# Autodesk Inventor assembly: Assembly11 (Cam Sub Assembly)
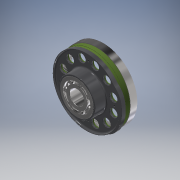
[picture p0: Inventor's stored thumbnail of the model, 180x180]
Saved by Autodesk Inventor 2018 (Build 220112000, 112)
## iProperties
Created: 2023-05-02
Part Number: Assembly11 (Cam Sub Assembly)
Document SubType Name: Assembly
Designer: Habib Mohamed
Author: Habib Mohamed
## Documents named in this file (6)
- D:\Inventor\My projects\Rotary Engine\Assembly\Assembly11 (Cam Sub Assembly).iam
- D:\Inventor\My projects\Rotary Engine\Component 18 (Front Cam Disc).ipt
- D:\Inventor\My projects\Rotary Engine\Component 19 (Rear Cam Disc).ipt
- D:\Inventor\My projects\Rotary Engine\Component 21 (Hollow Wheel).ipt
- C:\Users\Habib Mohamed\Documents\Inventor\Content Center Files\R2018\en-US\DIN 625 - T3\DIN 625 T3 - 4202 - 15 x 35 x 14.ipt
- C:\Users\Habib Mohamed\Documents\Inventor\Content Center Files\R2018\en-US\ISO 7046-1(2)\DIN EN ISO 7046-1 - M2 x 3 - 4.8 - Z.ipt
## Components (7 placed, 5 different names)
1. Component 18 (Front Cam Disc):1 — Mate:1, Mate:2, Mate:3, Mate:6
2. Component 19 (Rear Cam Disc):1 — Mate:1, Mate:2, Mate:3, Mate:4, Mate:5, Mate:7, Mate:8, Mate:9, Mate:10
3. Component 21 (Hollow Wheel):1 — Mate:4, Mate:5
4. DIN 625 - T3 4202 - 15 x 35 x 14:1 — Mate:6, Mate:7
5. DIN EN ISO 7046-1 Z M2 x 3 - 4.8 - Z:1 — Mate:8
6. DIN EN ISO 7046-1 Z M2 x 3 - 4.8 - Z:2 — Mate:9
7. DIN EN ISO 7046-1 Z M2 x 3 - 4.8 - Z:3 — Mate:10
## Relationships (10: Mate 10)
- Mate:1: Component 18 (Front Cam Disc):1 ↔ Component 19 (Rear Cam Disc):1
- Mate:2: Component 18 (Front Cam Disc):1 ↔ Component 19 (Rear Cam Disc):1
- Mate:3: Component 18 (Front Cam Disc):1 ↔ Component 19 (Rear Cam Disc):1
- Mate:4: Component 19 (Rear Cam Disc):1 ↔ Component 21 (Hollow Wheel):1
- Mate:5: Component 19 (Rear Cam Disc):1 ↔ Component 21 (Hollow Wheel):1
- Mate:6: Component 18 (Front Cam Disc):1 ↔ DIN 625 - T3 4202 - 15 x 35 x 14:1
- Mate:7: Component 19 (Rear Cam Disc):1 ↔ DIN 625 - T3 4202 - 15 x 35 x 14:1
- Mate:8: Component 19 (Rear Cam Disc):1 ↔ DIN EN ISO 7046-1 Z M2 x 3 - 4.8 - Z:1
- Mate:9: Component 19 (Rear Cam Disc):1 ↔ DIN EN ISO 7046-1 Z M2 x 3 - 4.8 - Z:2
- Mate:10: Component 19 (Rear Cam Disc):1 ↔ DIN EN ISO 7046-1 Z M2 x 3 - 4.8 - Z:3
